# Autodesk Inventor assembly: коробка + сервак
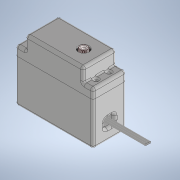
[picture p0: Inventor's stored thumbnail of the model, 180x180]
Saved by Autodesk Inventor 2021 (Build 250183000, 183)
## iProperties
Created: 2023-02-15
Part Number: коробка + сервак
Document SubType Name: Assembly
Designer: Tasya
Author: Tasya
## Documents named in this file (3)
- C:\Users\Tasya\Desktop\теплица\3D модели\Сборки iam\коробка + сервак.iam
- C:\Users\Tasya\Desktop\теплица\форточка\коробка сервак.ipt
- C:\Users\Tasya\Desktop\теплица\форточка\сервопривод.ipt
## Components (2 placed, 2 different names)
1. коробка сервак:1 — Совмещение:1, Совмещение:2, Совмещение:3, Совмещение:4
2. сервопривод:1 — Совмещение:1, Совмещение:2, Совмещение:3, Совмещение:4
## Relationships (4: Mate 4)
- Совмещение:1 [Mate] (2 mm): коробка сервак:1 ↔ сервопривод:1
- Совмещение:2 [Mate] (2 mm): коробка сервак:1 ↔ сервопривод:1
- Совмещение:3 [Mate]: коробка сервак:1 ↔ сервопривод:1
- Совмещение:4 [Mate]: коробка сервак:1 ↔ сервопривод:1
